# Autodesk Inventor assembly: BottomChassis
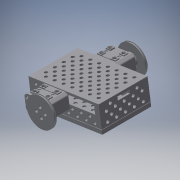
[picture p0: Inventor's stored thumbnail of the model, 180x180]
Saved by Autodesk Inventor 2016 (Build 200138000, 138)
## iProperties
Created: 2016-05-07
Part Number: BottomChassis
Document SubType Name: Assembly
Designer: mkepler
Author: mkepler
## Documents named in this file (5)
- C:\Users\mkepler\Google Drive\Michael Kepler\College\ECE\ECE 590\Final Project\Mechanical Design\Inventor Files\BottomChassis.iam
- C:\Users\mkepler\Google Drive\Michael Kepler\College\ECE\ECE 590\Final Project\Mechanical Design\Inventor Files\RaspPiCaseBottom.ipt
- C:\Users\mkepler\Google Drive\Michael Kepler\College\ECE\ECE 590\Final Project\Mechanical Design\Inventor Files\RaspPiCaseTop.ipt
- C:\Users\mkepler\Google Drive\Michael Kepler\College\ECE\ECE 590\Final Project\Mechanical Design\Inventor Files\xl320Servo.ipt
- C:\Users\mkepler\Google Drive\Michael Kepler\College\ECE\ECE 590\Final Project\Mechanical Design\Inventor Files\wheel.ipt
## Components (6 placed, 4 different names)
1. RaspPiCaseBottom:1 — Mate:1, Mate:2, Mate:3, Mate:4, Insert:1, Insert:2, Insert:3, Insert:4
2. RaspPiCaseTop:1 — Mate:1, Mate:2, Mate:3, Mate:4
3. xl320Servo:1 — Insert:1, Insert:2, Insert:5, Insert:6
4. xl320Servo:2 — Insert:3, Insert:4, Insert:7, Insert:8
5. wheel:1 — Insert:7, Insert:8
6. wheel:2 — Insert:5, Insert:6
## Relationships (12: Insert 8, Mate 4)
- Mate:1: RaspPiCaseBottom:1 ↔ RaspPiCaseTop:1
- Mate:2: RaspPiCaseBottom:1 ↔ RaspPiCaseTop:1
- Mate:3: RaspPiCaseBottom:1 ↔ RaspPiCaseTop:1
- Mate:4: RaspPiCaseBottom:1 ↔ RaspPiCaseTop:1
- Insert:1: RaspPiCaseBottom:1 ↔ xl320Servo:1
- Insert:2: RaspPiCaseBottom:1 ↔ xl320Servo:1
- Insert:3: RaspPiCaseBottom:1 ↔ xl320Servo:2
- Insert:4: RaspPiCaseBottom:1 ↔ xl320Servo:2
- Insert:5: xl320Servo:1 ↔ wheel:2
- Insert:6: xl320Servo:1 ↔ wheel:2
- Insert:7: xl320Servo:2 ↔ wheel:1
- Insert:8: xl320Servo:2 ↔ wheel:1
